# Autodesk Inventor assembly: McCrea_walle_jumper_walle
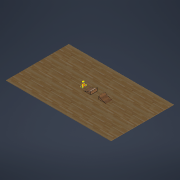
[picture p0: Inventor's stored thumbnail of the model, 180x180]
Saved by Autodesk Inventor 2022 (Build 260153000, 153)
## iProperties
Created: 2022-02-12
Part Number: McCrea_walle_jumper_walle
Document SubType Name: Assembly
Designer: MatusBarany
Author: MatusBarany
## Documents named in this file (4)
- C:\Users\MatusBarany\Documents\Inventor\wall-e\assembly\McCrea_walle_jumper_walle.iam
- C:\Users\MatusBarany\Documents\Inventor\wall-e\assembly\McCrea_WALLE_bez_HEAD_walle.iam
- C:\Users\MatusBarany\Documents\Inventor\wall-e\matus\plocha\McCrea_plocha_walle.ipt
- C:\Users\MatusBarany\Documents\Inventor\wall-e\matus\plocha\McCrea_rampa_walle.ipt
## Components (4 placed, 3 different names)
1. McCrea_WALLE_bez_HEAD_walle:1 [sub-assembly]
2. McCrea_plocha_walle:1 — Mate:1, Mate:2, Angle:1
3. McCrea_rampa_walle:1 — Mate:1, Flush:1
4. McCrea_rampa_walle:2 — Mate:2, Flush:1, Angle:1
## Relationships (4: Mate 2, Flush 1, Angle 1)
- Mate:1: McCrea_plocha_walle:1 ↔ McCrea_rampa_walle:1
- Mate:2: McCrea_plocha_walle:1 ↔ McCrea_rampa_walle:2
- Flush:1: McCrea_rampa_walle:1 ↔ McCrea_rampa_walle:2
- Angle:1 (90 deg): McCrea_plocha_walle:1 ↔ McCrea_rampa_walle:2
